# Autodesk Inventor assembly: Assembly2
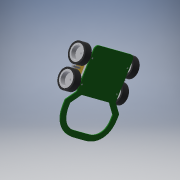
[picture p0: Inventor's stored thumbnail of the model, 180x180]
Saved by Autodesk Inventor 2016 (Build 200138000, 138)
## iProperties
Created: 2017-05-26
Part Number: Assembly2
Material: Ogólny
Document SubType Name: Assembly
Designer: Karol
Author: Karol
## Documents named in this file (14)
- D:\Git\MicromouseDixi\hardware\models\Dixi.iam
- D:\Git\MicromouseDixi\hardware\models\wheel.ipt
- D:\Git\MicromouseDixi\hardware\models\togh.ipt
- D:\Git\MicromouseDixi\hardware\models\bolt.ipt
- D:\Git\MicromouseDixi\hardware\models\tyre.ipt
- D:\Git\MicromouseDixi\hardware\models\magnet.ipt
- D:\Git\MicromouseDixi\hardware\models\mainpcb.ipt
- D:\ele\MicroMouse\v2\motor.ipt
- D:\Git\MicromouseDixi\hardware\models\bolt_MIR.ipt
- D:\Git\MicromouseDixi\hardware\models\wheel_MIR.ipt
- D:\Git\MicromouseDixi\hardware\models\magnet_MIR.ipt
- D:\Git\MicromouseDixi\hardware\models\togh_MIR5.ipt
- D:\Git\MicromouseDixi\hardware\models\tyre_MIR.ipt
- D:\ele\MicroMouse\v2\motor_MIR4.ipt
## Components (19 placed, 13 different names)
1. mainpcb:1 — Rigid:38, Rigid:52
2. bolt:3 — Rotational:1
3. bolt:4 — Rotational:19
4. wheel:3
5. wheel:4
6. magnet:4
7. togh:2 — Rotational:19, Rotational:1, Rigid:38, Rigid:39
8. tyre:3
9. tyre:4
10. motor:1 — Rigid:39
11. bolt_MIR:1 — Rigid:46, Rotational:23
12. bolt_MIR:2 — Rigid:47, Rigid:48, Rotational:22
13. wheel_MIR:1 — Rigid:46, Rigid:49
14. wheel_MIR:2 — Rigid:47, Rigid:50
15. magnet_MIR:1 — Rigid:48
16. togh_MIR5:1 — Rotational:22, Rotational:23, Rigid:51, Rigid:52
17. tyre_MIR:1 — Rigid:49
18. tyre_MIR:2 — Rigid:50
19. motor_MIR4:1 — Rigid:51
## Relationships (18: WeldJoint 14, RevoluteJoint 4)
- [WeldJoint]: bolt:4 ↔ wheel:4
- [WeldJoint]: bolt:3 ↔ wheel:3
- [WeldJoint]: bolt:4 ↔ magnet:4
- Rotational:19 [RevoluteJoint]: bolt:4 ↔ togh:2
- [WeldJoint]: wheel:3 ↔ tyre:3
- [WeldJoint]: wheel:4 ↔ tyre:4
- Rotational:1 [RevoluteJoint]: bolt:3 ↔ togh:2
- Rigid:38 [WeldJoint]: mainpcb:1 ↔ togh:2
- Rigid:39 [WeldJoint] (-0.5 mm): togh:2 ↔ motor:1
- Rigid:46 [WeldJoint]: bolt_MIR:1 ↔ wheel_MIR:1
- Rigid:47 [WeldJoint]: bolt_MIR:2 ↔ wheel_MIR:2
- Rigid:48 [WeldJoint]: bolt_MIR:2 ↔ magnet_MIR:1
- Rotational:22 [RevoluteJoint]: bolt_MIR:2 ↔ togh_MIR5:1
- Rotational:23 [RevoluteJoint]: bolt_MIR:1 ↔ togh_MIR5:1
- Rigid:49 [WeldJoint]: wheel_MIR:1 ↔ tyre_MIR:1
- Rigid:50 [WeldJoint]: wheel_MIR:2 ↔ tyre_MIR:2
- Rigid:51 [WeldJoint] (-0.5 mm): togh_MIR5:1 ↔ motor_MIR4:1
- Rigid:52 [WeldJoint] (1.4 mm): mainpcb:1 ↔ togh_MIR5:1
## Named parameters: d102_d99 = 0 mm, d105_d68 = 0 mm, d106_d67 = 0 mm, d107_d21 = -4.793458 deg, d108_d22 = -0.02503 mm, d111_d4 = 0 mm, d112_d5 = 0.127925 deg, d113_d6 = 0 mm, d114_d7 = -6.839272 deg, d117_d14 = 0 mm, d118_d15 = 2.56641 deg
